# Autodesk Inventor assembly: VITOOS AD5S LINK
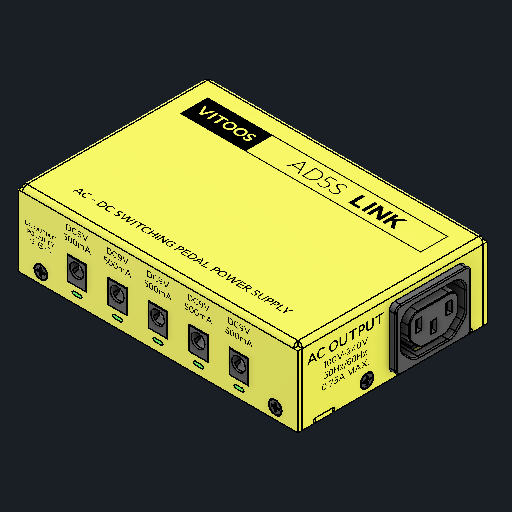
[picture p0: Inventor's stored thumbnail of the model, 512x512]
Saved by Autodesk Inventor 2026.2 (Build 302298000, 298)
## iProperties
Created: 2026-05-29
Part Number: VITOOS AD5S LINK
Document SubType Name: Assembly
Designer: JoshuaEah
Author: JoshuaEah
## Documents named in this file (8)
- C:\Users\JoshuaEah\Documents\GitHub\Designed-Trinkets\Guitar\Modular Pedalboard\Pedals\Power Supply\VITOOS AD5S LINK.iam
- C:\Users\JoshuaEah\Documents\GitHub\Designed-Trinkets\Guitar\Modular Pedalboard\Pedals\Power Supply\Components\Upper Case.ipt
- C:\Users\JoshuaEah\Documents\GitHub\Designed-Trinkets\Guitar\Modular Pedalboard\Pedals\Power Supply\Components\Lower Case.ipt
- C:\Users\JoshuaEah\Documents\GitHub\Designed-Trinkets\Guitar\Modular Pedalboard\Pedals\Power Supply\Components\DC Jack.ipt
- C:\Users\JoshuaEah\Documents\GitHub\Designed-Trinkets\Guitar\Modular Pedalboard\Pedals\Power Supply\Components\C14 Inlet.ipt
- C:\Users\JoshuaEah\Documents\GitHub\Designed-Trinkets\Guitar\Modular Pedalboard\Pedals\Power Supply\Components\C13 Inlet.ipt
- C:\Users\JoshuaEah\Documents\GitHub\Designed-Trinkets\Guitar\Modular Pedalboard\Pedals\Power Supply\Components\M3x4 FHCS.ipt
- C:\Users\JoshuaEah\Documents\GitHub\Designed-Trinkets\Guitar\Modular Pedalboard\Pedals\Power Supply\Components\Status Indicator.ipt
## Components (22 placed, 7 different names)
1. Upper Case:1 — Mate:1, Mate:3, Mate:2, Rigid:1, Slider:1, Mate:4, Insert:3, Insert:4, Insert:5, Insert:6, Insert:7, Insert:8, Insert:9, Insert:10, Mate:5, Mate:6, Flush:1, Insert:11, Insert:12, Insert:13, Insert:14, Insert:15
2. Lower Case:1 — Mate:1, Mate:3, Mate:2
3. C14 Inlet:1 — Slider:1, Mate:4
4. C13 Inlet:1 — Mate:5, Mate:6, Flush:1
5. M3x4 FHCS:1 — Insert:3
6. M3x4 FHCS:2 — Insert:4
7. M3x4 FHCS:3 — Insert:5
8. M3x4 FHCS:4 — Insert:6
9. M3x4 FHCS:5 — Insert:7
10. M3x4 FHCS:6 — Insert:8
11. M3x4 FHCS:7 — Insert:9
12. M3x4 FHCS:8 — Insert:10
13. Status Indicator:1 — Insert:11
14. Status Indicator:2 — Insert:12
15. Status Indicator:3 — Insert:13
16. Status Indicator:4 — Insert:14
17. Status Indicator:5 — Insert:15
18. DC Jack:1 — Rigid:1
19. DC Jack:2
20. DC Jack:3
21. DC Jack:4
22. DC Jack:5
## Component patterns: (5 elements, first: DC Jack:1)
## Relationships (22: Insert 13, Mate 6, WeldJoint 1, TranslationJoint 1, Flush 1)
- Mate:1: Upper Case:1 ↔ Lower Case:1
- Mate:3: Upper Case:1 ↔ Lower Case:1
- Mate:2: Upper Case:1 ↔ Lower Case:1
- Rigid:1 [WeldJoint]: Upper Case:1 ↔ DC Jack:1
- Slider:1 [TranslationJoint]: Upper Case:1 ↔ C14 Inlet:1
- Mate:4: Upper Case:1 ↔ C14 Inlet:1
- Insert:3: Upper Case:1 ↔ M3x4 FHCS:1
- Insert:4: Upper Case:1 ↔ M3x4 FHCS:2
- Insert:5: Upper Case:1 ↔ M3x4 FHCS:3
- Insert:6: Upper Case:1 ↔ M3x4 FHCS:4
- Insert:7: Upper Case:1 ↔ M3x4 FHCS:5
- Insert:8: Upper Case:1 ↔ M3x4 FHCS:6
- Insert:9: Upper Case:1 ↔ M3x4 FHCS:7
- Insert:10: Upper Case:1 ↔ M3x4 FHCS:8
- Mate:5: Upper Case:1 ↔ C13 Inlet:1
- Mate:6: Upper Case:1 ↔ C13 Inlet:1
- Flush:1: Upper Case:1 ↔ C13 Inlet:1
- Insert:11: Upper Case:1 ↔ Status Indicator:1
- Insert:12: Upper Case:1 ↔ Status Indicator:2
- Insert:13: Upper Case:1 ↔ Status Indicator:3
- Insert:14: Upper Case:1 ↔ Status Indicator:4
- Insert:15: Upper Case:1 ↔ Status Indicator:5
